# Autodesk Inventor assembly: ArticulatedIntake
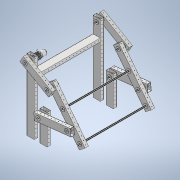
[picture p0: Inventor's stored thumbnail of the model, 180x180]
Saved by Autodesk Inventor 2022 (Build 260153000, 153)
## iProperties
Created: 2022-01-31
Part Number: ArticulatedIntake
Document SubType Name: Assembly
Designer: tagaz
Author: tagaz
## Documents named in this file (12)
- C:\Users\tagaz\OneDrive\Documents\T3-Cad\CAD\2022 Parts\Intake\ArticulatedIntake.iam
- C:\Users\tagaz\OneDrive\Documents\T3-Cad\CAD\2022 Parts\Intake\AIntakeVersa.ipt
- C:\Users\tagaz\OneDrive\Documents\T3-Cad\CAD\2022 Parts\Intake\AIntakeWheelShaft.ipt
- C:\Users\tagaz\OneDrive\Documents\T3-Cad\CAD\Bearing  for THUNDER.ipt
- C:\Users\tagaz\OneDrive\Documents\T3-Cad\CAD\2022 Parts\Intake\AIntakeSupport2.ipt
- C:\Users\tagaz\OneDrive\Documents\T3-Cad\CAD\2022 Parts\Intake\AIntakeSupport1.ipt
- C:\Users\tagaz\OneDrive\Documents\T3-Cad\CAD\2022 Parts\Intake\AIntakeArm1.ipt
- C:\Users\tagaz\OneDrive\Documents\T3-Cad\CAD\2022 Parts\Intake\AIntakeArm2.ipt
- C:\Users\tagaz\OneDrive\Documents\T3-Cad\CAD\2022 Parts\Intake\AIntakeArmShaft.ipt
- C:\Users\tagaz\OneDrive\Documents\T3-Cad\CAD\0.5in Hex Hub.ipt
- C:\Users\tagaz\OneDrive\Documents\T3-Cad\CAD\Generic and Stock\RevMotorParts\Neo550Assembly.iam
- C:\Users\tagaz\OneDrive\Documents\T3-Cad\CAD\2022 Parts\Intake\AIntakeSupport3.ipt
## Components (59 placed, 11 different names)
1. AIntakeVersa:1 — Flush:1, Flush:2, Mate:1, Mate:29, Mate:30, Mate:32, Insert:29, Insert:30, Insert:31, Insert:32, Insert:33, Insert:37, Insert:38, Insert:39
2. AIntakeVersa:2 — Flush:1, Flush:2, Mate:1, Mate:22, Mate:23, Mate:24, Mate:27, Insert:5, Insert:6, Insert:9, Insert:10, Insert:11, Insert:14, Insert:15, Insert:16
3. AIntakeSupport2:1 — Flush:5, Flush:6, Flush:7, Flush:9, Mate:4, Mate:5, Mate:21, Mate:26, Mate:52, Mate:53, Mate:54, Flush:22
4. AIntakeSupport2:2 — Flush:5, Flush:6, Flush:8, Flush:10, Mate:4, Mate:6, Mate:28, Insert:34, Insert:35, Flush:21
5. AIntakeSupport1:1 — Flush:7, Flush:9, Mate:5, Mate:25, Insert:12, Insert:13
6. AIntakeSupport1:2 — Flush:8, Flush:10, Mate:6, Mate:31, Mate:33, Insert:36, Insert:40
7. AIntakeArm1:1 — Mate:24, Mate:25, Mate:27, Insert:17, Insert:18, Insert:19, Insert:20
8. AIntakeArm1:2 — Mate:31, Mate:32, Mate:33, Insert:23, Insert:24, Insert:25, Insert:28
9. AIntakeArm2:1 — Mate:28, Mate:29, Mate:30, Insert:21, Insert:22, Insert:26, Insert:27
10. AIntakeArm2:2 — Mate:21, Mate:22, Mate:23, Mate:26, Insert:3, Insert:7, Insert:8, Mate:49, Mate:50, Mate:51
11. Bearing  for THUNDER:1 — Insert:16
12. Bearing  for THUNDER:2 — Insert:13
13. Bearing  for THUNDER:3 — Insert:12
14. Bearing  for THUNDER:4 — Insert:15, Mate:35, Flush:11
15. Bearing  for THUNDER:5 — Insert:14, Mate:34
16. Bearing  for THUNDER:6 — Insert:10
17. Bearing  for THUNDER:7 — Insert:11
18. Bearing  for THUNDER:8 — Insert:7
19. Bearing  for THUNDER:9 — Insert:9
20. Bearing  for THUNDER:10 — Insert:6
21. Bearing  for THUNDER:11 — Insert:8, Mate:38, Flush:14, Mate:39
22. Bearing  for THUNDER:12 — Insert:5
23. Bearing  for THUNDER:16 — Insert:3
24. Bearing  for THUNDER:17 — Insert:25
25. Bearing  for THUNDER:18 — Insert:23, Mate:47, Flush:19
26. Bearing  for THUNDER:19 — Insert:31
27. Bearing  for THUNDER:20 — Insert:28
28. Bearing  for THUNDER:21 — Insert:22, Mate:44, Mate:45, Flush:17
29. Bearing  for THUNDER:22 — Insert:20, Mate:42, Flush:16, Mate:43
30. Bearing  for THUNDER:23 — Insert:27
31. Bearing  for THUNDER:24 — Insert:30, Flush:12
32. Bearing  for THUNDER:25 — Insert:18, Mate:40, Mate:41, Flush:15
33. Bearing  for THUNDER:26 — Insert:34
34. Bearing  for THUNDER:27 — Insert:17
35. Bearing  for THUNDER:28 — Insert:35
36. Bearing  for THUNDER:29 — Insert:29
37. Bearing  for THUNDER:30 — Insert:19
38. Bearing  for THUNDER:31 — Insert:32
39. Bearing  for THUNDER:32 — Insert:26
40. Bearing  for THUNDER:33 — Insert:33
41. Bearing  for THUNDER:34 — Insert:24, Mate:48, Flush:20
42. Bearing  for THUNDER:35 — Insert:36
43. Bearing  for THUNDER:36 — Insert:21, Mate:46, Flush:18
44. Bearing  for THUNDER:39 — Insert:37
45. Bearing  for THUNDER:42 — Insert:39
46. Bearing  for THUNDER:43 — Insert:38
47. Bearing  for THUNDER:44 — Insert:40
48. AIntakeWheelShaft:1 — Mate:34, Flush:12
49. AIntakeWheelShaft:2 — Mate:35, Flush:11
50. AIntakeArmShaft:2 — Mate:38, Flush:14, Mate:39
51. AIntakeArmShaft:3 — Mate:40, Mate:41, Flush:15
52. AIntakeArmShaft:4 — Mate:42, Flush:16, Mate:43
53. AIntakeArmShaft:5 — Mate:44, Mate:45, Flush:17
54. AIntakeArmShaft:6 — Mate:46, Flush:18
55. AIntakeArmShaft:7 — Mate:47, Flush:19
56. AIntakeArmShaft:8 — Mate:48, Flush:20
57. 0.5in Hex Hub:1 — Mate:49, Mate:50, Mate:51
58. Neo550Assembly:1 [sub-assembly] — Mate:52, Mate:53
59. AIntakeSupport3:1 — Flush:21, Mate:54, Flush:22
## Relationships (92: Insert 37, Mate 36, Flush 19)
- Flush:1: AIntakeVersa:1 ↔ AIntakeVersa:2
- Flush:2: AIntakeVersa:1 ↔ AIntakeVersa:2
- Mate:1 (444.5 mm): AIntakeVersa:1 ↔ AIntakeVersa:2
- Flush:5: AIntakeSupport2:1 ↔ AIntakeSupport2:2
- Flush:6: AIntakeSupport2:1 ↔ AIntakeSupport2:2
- Flush:7: AIntakeSupport2:1 ↔ AIntakeSupport1:1
- Flush:8: AIntakeSupport2:2 ↔ AIntakeSupport1:2
- Flush:9: AIntakeSupport2:1 ↔ AIntakeSupport1:1
- Flush:10: AIntakeSupport2:2 ↔ AIntakeSupport1:2
- Mate:4 (444.5 mm): AIntakeSupport2:1 ↔ AIntakeSupport2:2
- Mate:5 (41.275 mm): AIntakeSupport2:1 ↔ AIntakeSupport1:1
- Mate:6 (41.275 mm): AIntakeSupport2:2 ↔ AIntakeSupport1:2
- Mate:21: AIntakeSupport2:1 ↔ AIntakeArm2:2
- Mate:22: AIntakeVersa:2 ↔ AIntakeArm2:2
- Mate:23 (12.7 mm): AIntakeVersa:2 ↔ AIntakeArm2:2
- Mate:24: AIntakeVersa:2 ↔ AIntakeArm1:1
- Mate:25: AIntakeSupport1:1 ↔ AIntakeArm1:1
- Mate:26 (12.7 mm): AIntakeSupport2:1 ↔ AIntakeArm2:2
- Mate:27 (12.7 mm): AIntakeVersa:2 ↔ AIntakeArm1:1
- Mate:28: AIntakeSupport2:2 ↔ AIntakeArm2:1
- Mate:29: AIntakeVersa:1 ↔ AIntakeArm2:1
- Mate:30 (12.7 mm): AIntakeVersa:1 ↔ AIntakeArm2:1
- Mate:31: AIntakeSupport1:2 ↔ AIntakeArm1:2
- Mate:32: AIntakeVersa:1 ↔ AIntakeArm1:2
- Mate:33 (12.7 mm): AIntakeSupport1:2 ↔ AIntakeArm1:2
- Insert:3: AIntakeArm2:2 ↔ Bearing  for THUNDER:16
- Insert:5: AIntakeVersa:2 ↔ Bearing  for THUNDER:12
- Insert:6: AIntakeVersa:2 ↔ Bearing  for THUNDER:10
- Insert:7: AIntakeArm2:2 ↔ Bearing  for THUNDER:8
- Insert:8: AIntakeArm2:2 ↔ Bearing  for THUNDER:11
- Insert:9: AIntakeVersa:2 ↔ Bearing  for THUNDER:9
- Insert:10: AIntakeVersa:2 ↔ Bearing  for THUNDER:6
- Insert:11: AIntakeVersa:2 ↔ Bearing  for THUNDER:7
- Insert:12: AIntakeSupport1:1 ↔ Bearing  for THUNDER:3
- Insert:13: AIntakeSupport1:1 ↔ Bearing  for THUNDER:2
- Insert:14: AIntakeVersa:2 ↔ Bearing  for THUNDER:5
- Insert:15: AIntakeVersa:2 ↔ Bearing  for THUNDER:4
- Insert:16: AIntakeVersa:2 ↔ Bearing  for THUNDER:1
- Insert:17: AIntakeArm1:1 ↔ Bearing  for THUNDER:27
- Insert:18: AIntakeArm1:1 ↔ Bearing  for THUNDER:25
- Insert:19: AIntakeArm1:1 ↔ Bearing  for THUNDER:30
- Insert:20: AIntakeArm1:1 ↔ Bearing  for THUNDER:22
- Insert:21: AIntakeArm2:1 ↔ Bearing  for THUNDER:36
- Insert:22: AIntakeArm2:1 ↔ Bearing  for THUNDER:21
- Insert:23: AIntakeArm1:2 ↔ Bearing  for THUNDER:18
- Insert:24: AIntakeArm1:2 ↔ Bearing  for THUNDER:34
- Insert:25: AIntakeArm1:2 ↔ Bearing  for THUNDER:17
- Insert:26: AIntakeArm2:1 ↔ Bearing  for THUNDER:32
- Insert:27: AIntakeArm2:1 ↔ Bearing  for THUNDER:23
- Insert:28: AIntakeArm1:2 ↔ Bearing  for THUNDER:20
- Insert:29: AIntakeVersa:1 ↔ Bearing  for THUNDER:29
- Insert:30: AIntakeVersa:1 ↔ Bearing  for THUNDER:24
- Insert:31: AIntakeVersa:1 ↔ Bearing  for THUNDER:19
- Insert:32: AIntakeVersa:1 ↔ Bearing  for THUNDER:31
- Insert:33: AIntakeVersa:1 ↔ Bearing  for THUNDER:33
- Insert:34: AIntakeSupport2:2 ↔ Bearing  for THUNDER:26
- Insert:35: AIntakeSupport2:2 ↔ Bearing  for THUNDER:28
- Insert:36: AIntakeSupport1:2 ↔ Bearing  for THUNDER:35
- Insert:37: AIntakeVersa:1 ↔ Bearing  for THUNDER:39
- Insert:38: AIntakeVersa:1 ↔ Bearing  for THUNDER:43
- Insert:39: AIntakeVersa:1 ↔ Bearing  for THUNDER:42
- Insert:40: AIntakeSupport1:2 ↔ Bearing  for THUNDER:44
- Mate:34: Bearing  for THUNDER:5 ↔ AIntakeWheelShaft:1
- Mate:35: Bearing  for THUNDER:4 ↔ AIntakeWheelShaft:2
- Flush:11 (9.525 mm): Bearing  for THUNDER:4 ↔ AIntakeWheelShaft:2
- Flush:12 (-9.525 mm): Bearing  for THUNDER:24 ↔ AIntakeWheelShaft:1
- Mate:38: Bearing  for THUNDER:11 ↔ AIntakeArmShaft:2
- Flush:14 (6.35 mm): Bearing  for THUNDER:11 ↔ AIntakeArmShaft:2
- Mate:39: Bearing  for THUNDER:11 ↔ AIntakeArmShaft:2
- Mate:40: Bearing  for THUNDER:25 ↔ AIntakeArmShaft:3
- Mate:41: Bearing  for THUNDER:25 ↔ AIntakeArmShaft:3
- Flush:15 (6.35 mm): Bearing  for THUNDER:25 ↔ AIntakeArmShaft:3
- Mate:42: Bearing  for THUNDER:22 ↔ AIntakeArmShaft:4
- Flush:16 (6.35 mm): Bearing  for THUNDER:22 ↔ AIntakeArmShaft:4
- Mate:43: Bearing  for THUNDER:22 ↔ AIntakeArmShaft:4
- Mate:44: Bearing  for THUNDER:21 ↔ AIntakeArmShaft:5
- Mate:45: Bearing  for THUNDER:21 ↔ AIntakeArmShaft:5
- Flush:17 (-6.35 mm): Bearing  for THUNDER:21 ↔ AIntakeArmShaft:5
- Mate:46: Bearing  for THUNDER:36 ↔ AIntakeArmShaft:6
- Flush:18 (-6.35 mm): Bearing  for THUNDER:36 ↔ AIntakeArmShaft:6
- Mate:47: Bearing  for THUNDER:18 ↔ AIntakeArmShaft:7
- Flush:19 (6.35 mm): Bearing  for THUNDER:18 ↔ AIntakeArmShaft:7
- Mate:48: Bearing  for THUNDER:34 ↔ AIntakeArmShaft:8
- Flush:20 (6.35 mm): Bearing  for THUNDER:34 ↔ AIntakeArmShaft:8
- Mate:49: AIntakeArm2:2 ↔ 0.5in Hex Hub:1
- Mate:50: AIntakeArm2:2 ↔ 0.5in Hex Hub:1
- Mate:51: AIntakeArm2:2 ↔ 0.5in Hex Hub:1
- Mate:52: AIntakeSupport2:1 ↔ Neo550Assembly:1
- Mate:53: AIntakeSupport2:1 ↔ Neo550Assembly:1
- Flush:21: AIntakeSupport2:2 ↔ AIntakeSupport3:1
- Mate:54: AIntakeSupport2:1 ↔ AIntakeSupport3:1
- Flush:22 (114.3 mm): AIntakeSupport2:1 ↔ AIntakeSupport3:1
